# Autodesk Inventor assembly: roller motor
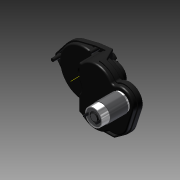
[picture p0: Inventor's stored thumbnail of the model, 180x180]
Saved by Autodesk Inventor 2011 (Build 150239000, 239)
## iProperties
Shininess: 64.0
Angle Display Precision: 2
Document Length Units: 11272
Document Angle Units: 11279
Document Time Units: 11290
Document Mass Units: 11286
Document Length Units Precision: 3
Document Angle Units Precision: 2
Category: Motors
Created: 2001-12-27
Document SubType Name: Assembly
Project: FIRST
Vendor: FisherPrice
Part Number: roller motor
Description: FisherPrice Motor and Gearbox
Density: 0.0
Volumn: 0.0
Area: 0.0
PropertySet Name: Model Information
Control State: 0
Master: False
Checked Out: False
Title: FisherPrice Motor and Gearbox
Author: Autodesk, Inc.
## Documents named in this file (4)
- R:\2012\Inventor\vkop\All_Motors\roller motor.iam
- R:\2012\Inventor\vkop\All_Motors\00968-9015_Housing2.ipt
- R:\2012\Inventor\vkop\All_Motors\00968-9015_Housing1.ipt
- R:\2012\Inventor\vkop\All_Motors\00968-9015_Spindle.ipt
## Components (3 placed, 3 different names)
1. 00968-9015_Housing2:1 — Flush:1, Flush:2, Mate:2, Mate:3
2. 00968-9015_Housing1:1 — Flush:1, Mate:1, Mate:2, Mate:3
3. 00968-9015_Spindle:1 — Flush:2, Mate:1
## Relationships (5: Mate 3, Flush 2)
- Flush:1: 00968-9015_Housing2:1 ↔ 00968-9015_Housing1:1
- Flush:2: 00968-9015_Housing2:1 ↔ 00968-9015_Spindle:1
- Mate:1: 00968-9015_Housing1:1 ↔ 00968-9015_Spindle:1
- Mate:2: 00968-9015_Housing2:1 ↔ 00968-9015_Housing1:1
- Mate:3: 00968-9015_Housing2:1 ↔ 00968-9015_Housing1:1
